# Autodesk Inventor assembly: Internal Rear Panels
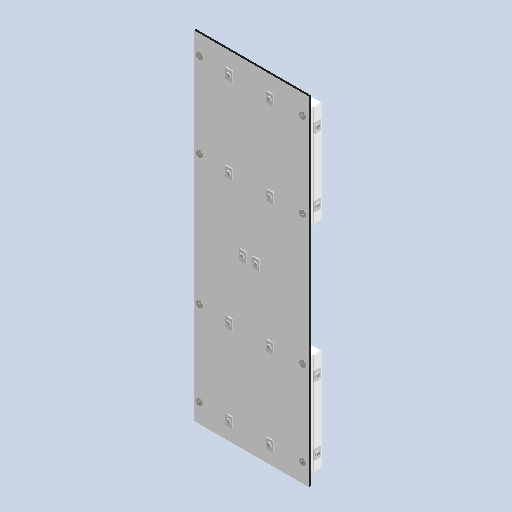
[picture p0: Inventor's stored thumbnail of the model, 512x512]
Saved by Autodesk Inventor 2024 (Build 280153000, 153)
## iProperties
Created: 2024-09-28
Part Number: Internal Rear Panels
Document SubType Name: Assembly
Designer: Ishaan
Author: Ishaan
## Documents named in this file (8)
- E:\Projects\Axiom--IDEX-3D-Printer\CAD\08 - Side Panelling\Internal Rear Panels.iam
- E:\Projects\Axiom--IDEX-3D-Printer\CAD\08 - Side Panelling\Rear Internal Side Panel.ipt
- E:\Projects\Axiom--IDEX-3D-Printer\CAD\00 - COTS Components\Hardware\Low Profile M5x16.ipt
- E:\Projects\Axiom--IDEX-3D-Printer\CAD\00 - COTS Components\Hardware\SHCSM5x8.ipt
- E:\Projects\Axiom--IDEX-3D-Printer\CAD\00 - COTS Components\Hardware\M5 T SLOT NUT.ipt
- E:\Projects\Axiom--IDEX-3D-Printer\CAD\08 - Side Panelling\Rear Side Panel Riser Bracket.ipt
- E:\Projects\Axiom--IDEX-3D-Printer\CAD\00 - COTS Components\Hardware\M5 LOCKNUT.ipt
- E:\Projects\Axiom--IDEX-3D-Printer\CAD\00 - COTS Components\Hardware\SHCSM5x16.ipt
## Components (57 placed, 7 different names)
1. Rear Internal Side Panel:1 — Insert:1, Insert:2, Insert:3, Insert:4, Insert:5, Insert:6, Insert:7, Insert:8, Insert:9, Insert:10, Insert:11, Insert:12, Insert:13, Insert:14, Insert:15, Insert:16, Insert:17, Insert:18, Insert:19, Insert:20, Insert:21, Insert:22, Insert:23, Insert:24, Insert:25, Insert:26, Insert:27, Insert:28, Angle:1, Angle:2, Angle:3, Angle:4, Angle:5, Angle:6, Angle:7, Angle:8, Angle:9, Angle:10, Insert:29, Insert:30, Insert:31, Insert:32, Insert:33, Insert:34, Insert:35, Insert:36, Angle:19, Angle:20, Angle:21, Angle:22, Angle:23, Angle:24, Angle:25, Angle:26
2. Low Profile M5x16:1 — Insert:1
3. Low Profile M5x16:2 — Insert:2
4. Low Profile M5x16:3 — Insert:3
5. Low Profile M5x16:4 — Insert:4
6. Low Profile M5x16:5 — Insert:5
7. Low Profile M5x16:6 — Insert:6
8. Low Profile M5x16:7 — Insert:7
9. Low Profile M5x16:8 — Insert:8
10. SHCSM5x8:1 — Insert:9
11. SHCSM5x8:2 — Insert:10
12. SHCSM5x8:3 — Insert:12
13. SHCSM5x8:4 — Insert:11
14. SHCSM5x8:5 — Insert:17
15. SHCSM5x8:6 — Insert:18
16. SHCSM5x8:7 — Insert:14
17. SHCSM5x8:8 — Insert:13
18. SHCSM5x8:9 — Insert:15
19. SHCSM5x8:10 — Insert:16
20. M5 T SLOT NUT:1 — Insert:19, Angle:1
21. M5 T SLOT NUT:2 — Insert:20, Angle:2
22. M5 T SLOT NUT:3 — Insert:21, Angle:6
23. M5 T SLOT NUT:4 — Insert:22, Angle:3
24. M5 T SLOT NUT:5 — Insert:23, Angle:5
25. M5 T SLOT NUT:6 — Insert:24, Angle:4
26. M5 T SLOT NUT:7 — Insert:26, Angle:7
27. M5 T SLOT NUT:8 — Insert:25, Angle:9
28. M5 T SLOT NUT:9 — Insert:27, Angle:8
29. M5 T SLOT NUT:10 — Insert:28, Angle:10
30. Rear Side Panel Riser Bracket:1 — Insert:31, Insert:32, Insert:39, Insert:40, Angle:13, Angle:14, Insert:47, Insert:48, Insert:57, Insert:58
31. Rear Side Panel Riser Bracket:2 — Insert:29, Insert:30, Insert:37, Insert:38, Angle:11, Angle:12, Insert:45, Insert:46, Insert:59, Insert:60
32. Rear Side Panel Riser Bracket:3 — Insert:35, Insert:36, Insert:43, Insert:44, Angle:17, Angle:18, Insert:49, Insert:50, Insert:55, Insert:56
33. Rear Side Panel Riser Bracket:4 — Insert:33, Insert:34, Insert:41, Insert:42, Angle:15, Angle:16, Insert:51, Insert:52, Insert:53, Insert:54
34. M5 LOCKNUT:1 — Insert:37, Angle:11
35. M5 LOCKNUT:2 — Insert:38, Angle:12
36. M5 LOCKNUT:3 — Insert:39, Angle:13
37. M5 LOCKNUT:4 — Insert:40, Angle:14
38. M5 LOCKNUT:5 — Insert:41, Angle:15
39. M5 LOCKNUT:6 — Insert:42, Angle:16
40. M5 LOCKNUT:7 — Insert:43, Angle:17
41. M5 LOCKNUT:8 — Insert:44, Angle:18
42. SHCSM5x16:1 — Insert:45
43. SHCSM5x16:2 — Insert:46
44. SHCSM5x16:3 — Insert:47
45. SHCSM5x16:4 — Insert:48
46. SHCSM5x16:5 — Insert:49
47. SHCSM5x16:6 — Insert:50
48. SHCSM5x16:7 — Insert:51
49. SHCSM5x16:8 — Insert:52
50. M5 T SLOT NUT:11 — Insert:53, Angle:19
51. M5 T SLOT NUT:12 — Insert:54, Angle:20
52. M5 T SLOT NUT:13 — Insert:55, Angle:21
53. M5 T SLOT NUT:14 — Insert:56, Angle:22
54. M5 T SLOT NUT:15 — Insert:57, Angle:23
55. M5 T SLOT NUT:16 — Insert:58, Angle:24
56. M5 T SLOT NUT:17 — Insert:59, Angle:25
57. M5 T SLOT NUT:18 — Insert:60, Angle:26
## Relationships (86: Insert 60, Angle 26)
- Insert:1: Rear Internal Side Panel:1 ↔ Low Profile M5x16:1
- Insert:2: Rear Internal Side Panel:1 ↔ Low Profile M5x16:2
- Insert:3: Rear Internal Side Panel:1 ↔ Low Profile M5x16:3
- Insert:4: Rear Internal Side Panel:1 ↔ Low Profile M5x16:4
- Insert:5: Rear Internal Side Panel:1 ↔ Low Profile M5x16:5
- Insert:6: Rear Internal Side Panel:1 ↔ Low Profile M5x16:6
- Insert:7: Rear Internal Side Panel:1 ↔ Low Profile M5x16:7
- Insert:8: Rear Internal Side Panel:1 ↔ Low Profile M5x16:8
- Insert:9: Rear Internal Side Panel:1 ↔ SHCSM5x8:1
- Insert:10: Rear Internal Side Panel:1 ↔ SHCSM5x8:2
- Insert:11: Rear Internal Side Panel:1 ↔ SHCSM5x8:4
- Insert:12: Rear Internal Side Panel:1 ↔ SHCSM5x8:3
- Insert:13: Rear Internal Side Panel:1 ↔ SHCSM5x8:8
- Insert:14: Rear Internal Side Panel:1 ↔ SHCSM5x8:7
- Insert:15: Rear Internal Side Panel:1 ↔ SHCSM5x8:9
- Insert:16: Rear Internal Side Panel:1 ↔ SHCSM5x8:10
- Insert:17: Rear Internal Side Panel:1 ↔ SHCSM5x8:5
- Insert:18: Rear Internal Side Panel:1 ↔ SHCSM5x8:6
- Insert:19 (2 mm): Rear Internal Side Panel:1 ↔ M5 T SLOT NUT:1
- Insert:20 (2 mm): Rear Internal Side Panel:1 ↔ M5 T SLOT NUT:2
- Insert:21 (2 mm): Rear Internal Side Panel:1 ↔ M5 T SLOT NUT:3
- Insert:22 (2 mm): Rear Internal Side Panel:1 ↔ M5 T SLOT NUT:4
- Insert:23 (2 mm): Rear Internal Side Panel:1 ↔ M5 T SLOT NUT:5
- Insert:24 (2 mm): Rear Internal Side Panel:1 ↔ M5 T SLOT NUT:6
- Insert:25 (2 mm): Rear Internal Side Panel:1 ↔ M5 T SLOT NUT:8
- Insert:26 (2 mm): Rear Internal Side Panel:1 ↔ M5 T SLOT NUT:7
- Insert:27 (2 mm): Rear Internal Side Panel:1 ↔ M5 T SLOT NUT:9
- Insert:28 (2 mm): Rear Internal Side Panel:1 ↔ M5 T SLOT NUT:10
- Angle:1 (0 deg): Rear Internal Side Panel:1 ↔ M5 T SLOT NUT:1
- Angle:2 (0 deg): Rear Internal Side Panel:1 ↔ M5 T SLOT NUT:2
- Angle:3 (0 deg): Rear Internal Side Panel:1 ↔ M5 T SLOT NUT:4
- Angle:4 (0 deg): Rear Internal Side Panel:1 ↔ M5 T SLOT NUT:6
- Angle:5 (0 deg): Rear Internal Side Panel:1 ↔ M5 T SLOT NUT:5
- Angle:6 (0 deg): Rear Internal Side Panel:1 ↔ M5 T SLOT NUT:3
- Angle:7 (0 deg): Rear Internal Side Panel:1 ↔ M5 T SLOT NUT:7
- Angle:8 (0 deg): Rear Internal Side Panel:1 ↔ M5 T SLOT NUT:9
- Angle:9 (0 deg): Rear Internal Side Panel:1 ↔ M5 T SLOT NUT:8
- Angle:10 (0 deg): Rear Internal Side Panel:1 ↔ M5 T SLOT NUT:10
- Insert:29: Rear Internal Side Panel:1 ↔ Rear Side Panel Riser Bracket:2
- Insert:30: Rear Internal Side Panel:1 ↔ Rear Side Panel Riser Bracket:2
- Insert:31: Rear Internal Side Panel:1 ↔ Rear Side Panel Riser Bracket:1
- Insert:32: Rear Internal Side Panel:1 ↔ Rear Side Panel Riser Bracket:1
- Insert:33: Rear Internal Side Panel:1 ↔ Rear Side Panel Riser Bracket:4
- Insert:34: Rear Internal Side Panel:1 ↔ Rear Side Panel Riser Bracket:4
- Insert:35: Rear Internal Side Panel:1 ↔ Rear Side Panel Riser Bracket:3
- Insert:36: Rear Internal Side Panel:1 ↔ Rear Side Panel Riser Bracket:3
- Insert:37: Rear Side Panel Riser Bracket:2 ↔ M5 LOCKNUT:1
- Insert:38: Rear Side Panel Riser Bracket:2 ↔ M5 LOCKNUT:2
- Insert:39: Rear Side Panel Riser Bracket:1 ↔ M5 LOCKNUT:3
- Insert:40: Rear Side Panel Riser Bracket:1 ↔ M5 LOCKNUT:4
- Insert:41: Rear Side Panel Riser Bracket:4 ↔ M5 LOCKNUT:5
- Insert:42: Rear Side Panel Riser Bracket:4 ↔ M5 LOCKNUT:6
- Insert:43: Rear Side Panel Riser Bracket:3 ↔ M5 LOCKNUT:7
- Insert:44: Rear Side Panel Riser Bracket:3 ↔ M5 LOCKNUT:8
- Angle:11 (0 deg): Rear Side Panel Riser Bracket:2 ↔ M5 LOCKNUT:1
- Angle:12 (0 deg): Rear Side Panel Riser Bracket:2 ↔ M5 LOCKNUT:2
- Angle:13 (0 deg): Rear Side Panel Riser Bracket:1 ↔ M5 LOCKNUT:3
- Angle:14 (0 deg): Rear Side Panel Riser Bracket:1 ↔ M5 LOCKNUT:4
- Angle:15 (0 deg): Rear Side Panel Riser Bracket:4 ↔ M5 LOCKNUT:5
- Angle:16 (0 deg): Rear Side Panel Riser Bracket:4 ↔ M5 LOCKNUT:6
- Angle:17 (0 deg): Rear Side Panel Riser Bracket:3 ↔ M5 LOCKNUT:7
- Angle:18 (0 deg): Rear Side Panel Riser Bracket:3 ↔ M5 LOCKNUT:8
- Insert:45: Rear Side Panel Riser Bracket:2 ↔ SHCSM5x16:1
- Insert:46: Rear Side Panel Riser Bracket:2 ↔ SHCSM5x16:2
- Insert:47: Rear Side Panel Riser Bracket:1 ↔ SHCSM5x16:3
- Insert:48: Rear Side Panel Riser Bracket:1 ↔ SHCSM5x16:4
- Insert:49: Rear Side Panel Riser Bracket:3 ↔ SHCSM5x16:5
- Insert:50: Rear Side Panel Riser Bracket:3 ↔ SHCSM5x16:6
- Insert:51: Rear Side Panel Riser Bracket:4 ↔ SHCSM5x16:7
- Insert:52: Rear Side Panel Riser Bracket:4 ↔ SHCSM5x16:8
- Insert:53 (2 mm): Rear Side Panel Riser Bracket:4 ↔ M5 T SLOT NUT:11
- Insert:54 (2 mm): Rear Side Panel Riser Bracket:4 ↔ M5 T SLOT NUT:12
- Insert:55 (2 mm): Rear Side Panel Riser Bracket:3 ↔ M5 T SLOT NUT:13
- Insert:56 (2 mm): Rear Side Panel Riser Bracket:3 ↔ M5 T SLOT NUT:14
- Insert:57 (2 mm): Rear Side Panel Riser Bracket:1 ↔ M5 T SLOT NUT:15
- Insert:58 (2 mm): Rear Side Panel Riser Bracket:1 ↔ M5 T SLOT NUT:16
- Insert:59 (2 mm): Rear Side Panel Riser Bracket:2 ↔ M5 T SLOT NUT:17
- Insert:60 (2 mm): Rear Side Panel Riser Bracket:2 ↔ M5 T SLOT NUT:18
- Angle:19 (0 deg): Rear Internal Side Panel:1 ↔ M5 T SLOT NUT:11
- Angle:20 (0 deg): Rear Internal Side Panel:1 ↔ M5 T SLOT NUT:12
- Angle:21 (0 deg): Rear Internal Side Panel:1 ↔ M5 T SLOT NUT:13
- Angle:22 (0 deg): Rear Internal Side Panel:1 ↔ M5 T SLOT NUT:14
- Angle:23 (0 deg): Rear Internal Side Panel:1 ↔ M5 T SLOT NUT:15
- Angle:24 (0 deg): Rear Internal Side Panel:1 ↔ M5 T SLOT NUT:16
- Angle:25 (0 deg): Rear Internal Side Panel:1 ↔ M5 T SLOT NUT:17
- Angle:26 (0 deg): Rear Internal Side Panel:1 ↔ M5 T SLOT NUT:18
